# Autodesk Inventor assembly: GameBoy
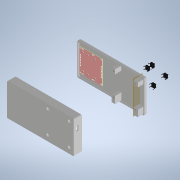
[picture p0: Inventor's stored thumbnail of the model, 180x180]
Saved by Autodesk Inventor 2022 (Build 260153000, 153)
## iProperties
Created: 2023-09-02
Part Number: GameBoy
Document SubType Name: Assembly
Designer: Petr Černý
Author: Petr Černý
## Documents named in this file (8)
- C:\Projekty\GameBoy\Enclosure_3D\3D Model\GameBoy.iam
- C:\Projekty\GameBoy\Enclosure_3D\3D Model\LowerHalf.ipt
- C:\Projekty\GameBoy\Enclosure_3D\3D Model\Upper_Half.ipt
- C:\Projekty\GameBoy\Enclosure_3D\3D Model\GameBoy_PCB.iam
- C:\Projekty\GameBoy\Enclosure_3D\3D Model\Nokia5110.iam
- C:\Projekty\GameBoy\Enclosure_3D\3D Model\Tactile_Push_Button.ipt
- C:\Projekty\GameBoy\Enclosure_3D\3D Model\3x AAA battery holder_update.iam
- C:\Projekty\GameBoy\Enclosure_3D\3D Model\BatteryDoor.ipt
## Components (11 placed, 7 different names)
1. LowerHalf:1 — Flush:9, Flush:10, Mate:12, Mate:13, Mate:31, Mate:33, Mate:34, Mate:35, Mate:36, Mate:37
2. Upper_Half:1 — Mate:5, Mate:6, Flush:9, Flush:10, Flush:11, Mate:32
3. GameBoy_PCB:1 [sub-assembly] — Mate:36, Mate:37
4. Nokia5110:1 [sub-assembly] — Mate:5, Mate:6, Mate:32
5. Tactile_Push_Button:1
6. Tactile_Push_Button:2
7. Tactile_Push_Button:3
8. Tactile_Push_Button:4
9. 3x AAA battery holder_update:1 [sub-assembly] — Mate:12, Mate:13, Mate:31
10. Tactile_Push_Button:5
11. BatteryDoor:1 — Mate:33, Mate:34, Mate:35
## Relationships (14: Mate 11, Flush 3)
- Mate:5: Upper_Half:1 ↔ Nokia5110:1
- Mate:6: Upper_Half:1 ↔ Nokia5110:1
- Flush:9: LowerHalf:1 ↔ Upper_Half:1
- Flush:10: LowerHalf:1 ↔ Upper_Half:1
- Flush:11 (-10 mm): Upper_Half:1
- Mate:12: LowerHalf:1 ↔ 3x AAA battery holder_update:1
- Mate:13 (5 mm): LowerHalf:1 ↔ 3x AAA battery holder_update:1
- Mate:31 (7.5 mm): LowerHalf:1 ↔ 3x AAA battery holder_update:1
- Mate:32: Upper_Half:1 ↔ Nokia5110:1
- Mate:33: LowerHalf:1 ↔ BatteryDoor:1
- Mate:34: LowerHalf:1 ↔ BatteryDoor:1
- Mate:35: LowerHalf:1 ↔ BatteryDoor:1
- Mate:36: LowerHalf:1 ↔ GameBoy_PCB:1
- Mate:37: LowerHalf:1 ↔ GameBoy_PCB:1
